# Autodesk Inventor assembly: imu_house_assembly
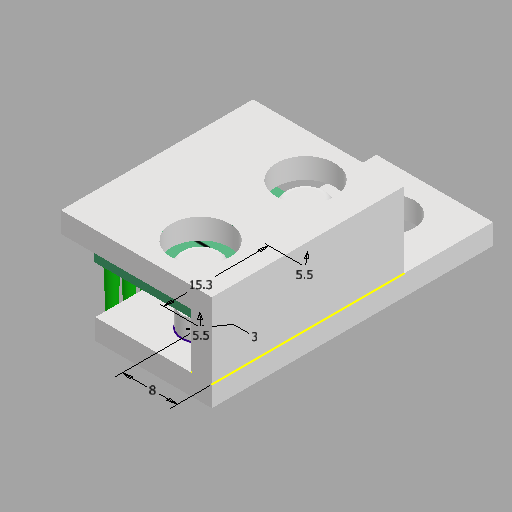
[picture p0: Inventor's stored thumbnail of the model, 512x512]
Saved by Autodesk Inventor 2025.2 (Build 292293000, 293)
## iProperties
Created: 2025-02-13
Part Number: imu_house_assembly
Document SubType Name: Assembly
Designer: Alex
Author: Alex
## Documents named in this file (4)
- C:\Shared\alex-bartella-schoolwork\4tb6\4tb6-repo\CAD_Model\thigh_mount_2\thigh_mount_2\imu_house_assembly.iam
- C:\Shared\alex-bartella-schoolwork\4tb6\4tb6-repo\CAD_Model\thigh_mount_2\thigh_mount_2\IMU_temp.ipt
- C:\Shared\alex-bartella-schoolwork\4tb6\4tb6-repo\CAD_Model\thigh_mount_2\thigh_mount_2\imu_housing_op.ipt
- C:\Shared\alex-bartella-schoolwork\4tb6\4tb6-repo\CAD_Model\thigh_mount_2\thigh_mount_2\imu screws.ipt
## Components (4 placed, 3 different names)
1. IMU_temp:1 — Mate:4, Mate:5, Mate:6, Mate:10, Mate:11
2. imu_housing_op:1 — Mate:6, Mate:8, Mate:9, Mate:11
3. imu screws:1 — Mate:4, Mate:5, Mate:8
4. imu screws:2 — Mate:9, Mate:10
## Relationships (7: Mate 7)
- Mate:4: IMU_temp:1 ↔ imu screws:1
- Mate:5: IMU_temp:1 ↔ imu screws:1
- Mate:6: IMU_temp:1 ↔ imu_housing_op:1
- Mate:8: imu_housing_op:1 ↔ imu screws:1
- Mate:9: imu_housing_op:1 ↔ imu screws:2
- Mate:10: IMU_temp:1 ↔ imu screws:2
- Mate:11: IMU_temp:1 ↔ imu_housing_op:1
